# Autodesk Inventor assembly: batteryCellAssembly
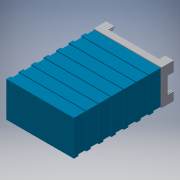
[picture p0: Inventor's stored thumbnail of the model, 180x180]
Saved by Autodesk Inventor 2019 (Build 230136000, 136)
## iProperties
Created: 2019-10-14
Part Number: batteryCellAssembly
Document SubType Name: Assembly
Designer: lagrecat
Author: lagrecat
## Documents named in this file (3)
- P:\me_fsae\2019-2020\TSV\octoberProtoypeParts\batteryCellAssembly.iam
- P:\me_fsae\2019-2020\TSV\octoberProtoypeParts\2018Parts\batteryCell.ipt
- P:\me_fsae\2019-2020\TSV\octoberProtoypeParts\2018Parts\batteryCellTop.ipt
## Components (2 placed, 2 different names)
1. batteryCell:1 — Mate:1, Flush:1, Flush:2
2. batteryCellTop:1 — Mate:1, Flush:1, Flush:2
## Relationships (3: Flush 2, Mate 1)
- Mate:1: batteryCell:1 ↔ batteryCellTop:1
- Flush:1: batteryCell:1 ↔ batteryCellTop:1
- Flush:2: batteryCell:1 ↔ batteryCellTop:1
